# Autodesk Inventor assembly: inner_uper_glide_assembly
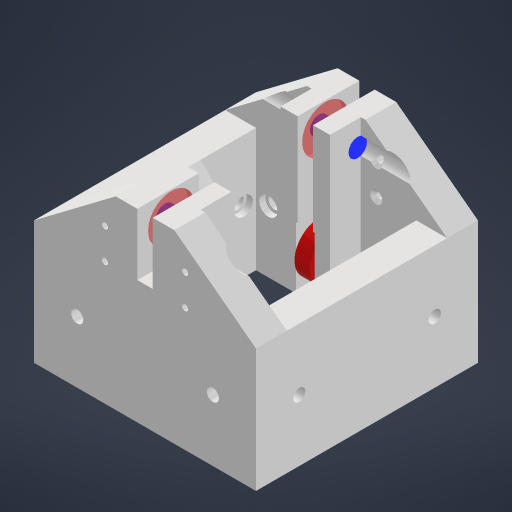
[picture p0: Inventor's stored thumbnail of the model, 512x512]
Saved by Autodesk Inventor 2024 (Build 280153000, 153)
## iProperties
Created: 2023-05-23
Part Number: inner_uper_glide_assembly
Document SubType Name: Assembly
Designer: aasmu
Author: aasmu
## Documents named in this file (5)
- C:\Users\aasmu\Documents\standing_desk\inner_uper_glide_assembly.iam
- C:\Users\aasmu\Documents\standing_desk\top_inner_glide_cartrige.ipt
- C:\Users\aasmu\Documents\standing_desk\cable_roller.ipt
- C:\Users\aasmu\Documents\standing_desk\roller_shaft.ipt
- C:\Users\aasmu\Documents\standing_desk\load_bearing.ipt
## Components (9 placed, 4 different names)
1. top_inner_glide_cartrige:1 — Rotational:1, Rotational:2, Rotational:3, Rotational:4, Rotational:5, Rotational:6
2. cable_roller:1 — Cylindrical:1
3. cable_roller:2 — Cylindrical:2
4. roller_shaft:1 — Cylindrical:1, Rotational:2
5. roller_shaft:2 — Cylindrical:2, Rotational:1
6. load_bearing:1 — Rotational:6
7. load_bearing:2 — Rotational:5
8. load_bearing:3 — Rotational:4
9. load_bearing:4 — Rotational:3
## Relationships (8: RevoluteJoint 6, CylindricalJoint 2)
- Cylindrical:1: cable_roller:1 ↔ roller_shaft:1
- Cylindrical:2: cable_roller:2 ↔ roller_shaft:2
- Rotational:1 [RevoluteJoint]: top_inner_glide_cartrige:1 ↔ roller_shaft:2
- Rotational:2 [RevoluteJoint]: top_inner_glide_cartrige:1 ↔ roller_shaft:1
- Rotational:3 [RevoluteJoint]: top_inner_glide_cartrige:1 ↔ load_bearing:4
- Rotational:4 [RevoluteJoint]: top_inner_glide_cartrige:1 ↔ load_bearing:3
- Rotational:5 [RevoluteJoint]: top_inner_glide_cartrige:1 ↔ load_bearing:2
- Rotational:6 [RevoluteJoint]: top_inner_glide_cartrige:1 ↔ load_bearing:1
